# Autodesk Inventor assembly: Servo Motor MG996R  With Attachments
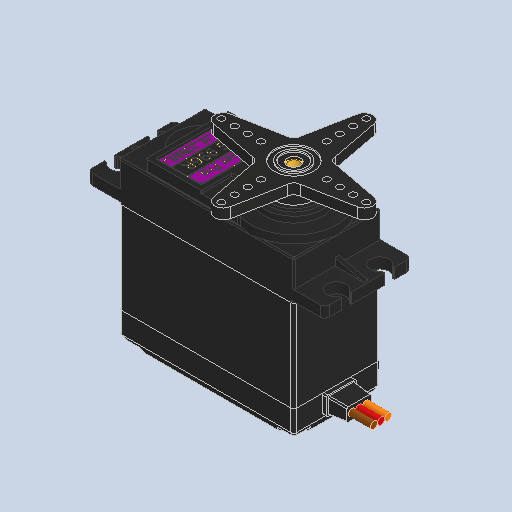
[picture p0: Inventor's stored thumbnail of the model, 512x512]
Saved by Autodesk Inventor 2023 (Build 270158000, 158)
## iProperties
Created: 2023-10-04
Part Number: Servo Motor MG996R  With Attachments
Document SubType Name: Assembly
Designer: zskus
Sending System: SOLIDWORKS 2016-2016040
MC: AMD64
MC_MODEL: Intel64 Family 6 Model 60 Stepping 3, GenuineIntel
OS: Windows_NT
FRU: Parasolid Version 28.0, build 204, 11- 9-2015
FORMAT: text
GUISE: transmit
KEY: Servo Motor MG996R  With Attachments
FILE: Servo Motor MG996R  With Attachments.x_t
DATE: Tue Oct 27 20:35:35 2020
Author: zskus
## Documents named in this file (14)
- C:\Users\zskus\Desktop\Folders\Personal Projects\Inventor\Project_1_Scooter\Parts\Servo Motor MG996R  With Attachments.iam
- C:\Users\zskus\Desktop\Folders\Personal Projects\Inventor\Project_1_Scooter\Parts\servoMotorMG996R.ipt
- C:\Users\zskus\Desktop\Folders\Personal Projects\Inventor\Project_1_Scooter\Parts\servoMotorMG996R_1.ipt
- C:\Users\zskus\Desktop\Folders\Personal Projects\Inventor\Project_1_Scooter\Parts\servoMotorMG996R_2.ipt
- C:\Users\zskus\Desktop\Folders\Personal Projects\Inventor\Project_1_Scooter\Parts\servoMotorMG996R_3.ipt
- C:\Users\zskus\Desktop\Folders\Personal Projects\Inventor\Project_1_Scooter\Parts\servoMotorMG996R_4.ipt
- C:\Users\zskus\Desktop\Folders\Personal Projects\Inventor\Project_1_Scooter\Parts\servoMotorMG996R_5.ipt
- C:\Users\zskus\Desktop\Folders\Personal Projects\Inventor\Project_1_Scooter\Parts\servoMotorMG996R_6.ipt
- C:\Users\zskus\Desktop\Folders\Personal Projects\Inventor\Project_1_Scooter\Parts\servoMotorMG996R_7.ipt
- C:\Users\zskus\Desktop\Folders\Personal Projects\Inventor\Project_1_Scooter\Parts\attachmentCircular.ipt
- C:\Users\zskus\Desktop\Folders\Personal Projects\Inventor\Project_1_Scooter\Parts\attachmentCircular_1.ipt
- C:\Users\zskus\Desktop\Folders\Personal Projects\Inventor\Project_1_Scooter\Parts\attachmentCross.ipt
- C:\Users\zskus\Desktop\Folders\Personal Projects\Inventor\Project_1_Scooter\Parts\attachmentStar.ipt
- C:\Users\zskus\Desktop\Folders\Personal Projects\Inventor\Project_1_Scooter\Parts\attachmentStraight.ipt
## Components (13 placed, 13 different names)
1. servoMotorMG996R — Flush:1, Flush:2, Mate:2, Flush:3, Flush:4, Mate:6
2. servoMotorMG996R_1 — Flush:3, Flush:4, Mate:6
3. servoMotorMG996R_2
4. servoMotorMG996R_3
5. servoMotorMG996R_4
6. servoMotorMG996R_5
7. servoMotorMG996R_6 — Mate:1, Mate:3, Mate:4, Mate:8
8. servoMotorMG996R_7 — Flush:1, Flush:2, Mate:2, Mate:3, Mate:4, Mate:5, Mate:7
9. attachmentCircular
10. attachmentCircular_1
11. attachmentCross — Mate:7, Mate:8
12. attachmentStar
13. attachmentStraight — Mate:1, Mate:5
## Relationships (12: Mate 8, Flush 4)
- Mate:1: servoMotorMG996R_6 ↔ attachmentStraight
- Flush:1: servoMotorMG996R ↔ servoMotorMG996R_7
- Flush:2: servoMotorMG996R ↔ servoMotorMG996R_7
- Mate:2: servoMotorMG996R ↔ servoMotorMG996R_7
- Mate:3: servoMotorMG996R_6 ↔ servoMotorMG996R_7
- Mate:4: servoMotorMG996R_6 ↔ servoMotorMG996R_7
- Mate:5: servoMotorMG996R_7 ↔ attachmentStraight
- Flush:3: servoMotorMG996R ↔ servoMotorMG996R_1
- Flush:4: servoMotorMG996R ↔ servoMotorMG996R_1
- Mate:6: servoMotorMG996R ↔ servoMotorMG996R_1
- Mate:7: servoMotorMG996R_7 ↔ attachmentCross
- Mate:8: servoMotorMG996R_6 ↔ attachmentCross
